# Autodesk Inventor assembly: Box Arm
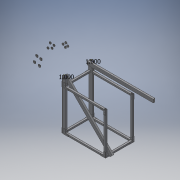
[picture p0: Inventor's stored thumbnail of the model, 180x180]
Saved by Autodesk Inventor 2018 (Build 220112000, 112)
## iProperties
Created: 2019-01-16
Part Number: Box Arm
Document SubType Name: Assembly
Designer: Gabriel
Author: Gabriel
## Documents named in this file (9)
- C:\Users\Gabriel\Documents\Drivebase Box Arm\Box Arm.iam
- C:\Users\Gabriel\Documents\Drivebase Box Arm\30in 1x1 Beam.ipt
- C:\Users\Gabriel\Documents\Drivebase Box Arm\25in 1x1 Beam.ipt
- C:\Users\Gabriel\Documents\Drivebase Box Arm\17in 1x1 Beam.ipt
- C:\Users\Gabriel\Documents\Drivebase Box Arm\23in 1x1 Beam.ipt
- C:\Users\Gabriel\Documents\Drivebase Box Arm\L gusset.ipt
- C:\Users\Gabriel\Documents\Drivebase Box Arm\34.48in Arm Bea.ipt
- C:\Users\Gabriel\Downloads\0_500_ID_x_1_125_OD_x_0_313_WD_Flanged_Bearing_217-2731.ipt
- C:\Users\Gabriel\Downloads\12t_Aluminum_Hub_Sprocket_35_Chain_1_2_Hex_Bore_217-2662.ipt
## Components (39 placed, 9 different names)
1. 30in 1x1 Beam:1 — Mate:13, Mate:14, Mate:37, Mate:38, Mate:74, Mate:75, Mate:81
2. 30in 1x1 Beam:2 — Mate:11, Mate:12, Mate:39, Mate:40, Mate:73, Mate:76, Mate:82
3. 25in 1x1 Beam:1 — Mate:57, Mate:58, Mate:59, Mate:60, Mate:65, Mate:66
4. 25in 1x1 Beam:2 — Mate:61, Mate:62, Mate:63, Mate:64, Mate:67, Mate:68
5. 25in 1x1 Beam:3 — Mate:29, Mate:30, Mate:53, Mate:54
6. 25in 1x1 Beam:4 — Mate:31, Mate:32, Mate:55, Mate:56
7. 17in 1x1 Beam:1 — Mate:69, Mate:70, Mate:71, Mate:72
8. 17in 1x1 Beam:2 — Mate:21, Mate:22, Mate:23, Mate:24
9. 23in 1x1 Beam:1 — Mate:43, Mate:44, Mate:49, Mate:50
10. 23in 1x1 Beam:2 — Mate:47, Mate:48, Mate:51, Mate:52
11. L gusset:1 — Mate:53, Mate:54, Mate:63, Mate:64
12. L gusset:4 — Mate:49, Mate:50, Mate:61, Mate:62
13. L gusset:5 — Mate:51, Mate:52, Mate:57, Mate:58
14. L gusset:7 — Mate:11, Mate:12, Mate:23, Mate:24
15. L gusset:9 — Mate:13, Mate:14, Mate:21, Mate:22
16. L gusset:11 — Mate:31, Mate:32, Mate:74, Mate:75
17. L gusset:12 — Mate:29, Mate:30, Mate:73, Mate:76
18. L gusset:13 — Mate:43, Mate:44
19. L gusset:14 — Mate:47, Mate:48
20. L gusset:15 — Mate:39, Mate:40, Mate:77, Mate:80
21. L gusset:16 — Mate:37, Mate:38, Mate:78, Mate:79
22. L gusset:17 — Mate:55, Mate:56, Mate:59, Mate:60
23. L gusset:18 — Mate:67, Mate:68, Mate:69, Mate:70
24. L gusset:19 — Mate:65, Mate:66, Mate:71, Mate:72
25. 34.48in Arm Beam:1 — Mate:82
26. 17in 1x1 Beam:3 — Mate:77, Mate:78, Mate:79, Mate:80
27. 34.48in Arm Bea:2 — Mate:81
28. 0_500_ID_x_1_125_OD_x_0_313_WD_Flanged_Bearing_217-2731:1
29. 0_500_ID_x_1_125_OD_x_0_313_WD_Flanged_Bearing_217-2731:2
30. 0_500_ID_x_1_125_OD_x_0_313_WD_Flanged_Bearing_217-2731:3
31. 0_500_ID_x_1_125_OD_x_0_313_WD_Flanged_Bearing_217-2731:4
32. 0_500_ID_x_1_125_OD_x_0_313_WD_Flanged_Bearing_217-2731:5
33. 0_500_ID_x_1_125_OD_x_0_313_WD_Flanged_Bearing_217-2731:6
34. 0_500_ID_x_1_125_OD_x_0_313_WD_Flanged_Bearing_217-2731:7
35. 0_500_ID_x_1_125_OD_x_0_313_WD_Flanged_Bearing_217-2731:8
36. 12t_Aluminum_Hub_Sprocket_35_Chain_1_2_Hex_Bore_217-2662:1
37. 12t_Aluminum_Hub_Sprocket_35_Chain_1_2_Hex_Bore_217-2662:2
38. 12t_Aluminum_Hub_Sprocket_35_Chain_1_2_Hex_Bore_217-2662:3
39. 12t_Aluminum_Hub_Sprocket_35_Chain_1_2_Hex_Bore_217-2662:4
## Relationships (54: Mate 54)
- Mate:11: 30in 1x1 Beam:2 ↔ L gusset:7
- Mate:12: 30in 1x1 Beam:2 ↔ L gusset:7
- Mate:13: 30in 1x1 Beam:1 ↔ L gusset:9
- Mate:14: 30in 1x1 Beam:1 ↔ L gusset:9
- Mate:21: 17in 1x1 Beam:2 ↔ L gusset:9
- Mate:22: 17in 1x1 Beam:2 ↔ L gusset:9
- Mate:23: 17in 1x1 Beam:2 ↔ L gusset:7
- Mate:24: 17in 1x1 Beam:2 ↔ L gusset:7
- Mate:29: 25in 1x1 Beam:3 ↔ L gusset:12
- Mate:30: 25in 1x1 Beam:3 ↔ L gusset:12
- Mate:31: 25in 1x1 Beam:4 ↔ L gusset:11
- Mate:32: 25in 1x1 Beam:4 ↔ L gusset:11
- Mate:37: 30in 1x1 Beam:1 ↔ L gusset:16
- Mate:38: 30in 1x1 Beam:1 ↔ L gusset:16
- Mate:39: 30in 1x1 Beam:2 ↔ L gusset:15
- Mate:40: 30in 1x1 Beam:2 ↔ L gusset:15
- Mate:43: 23in 1x1 Beam:1 ↔ L gusset:13
- Mate:44: 23in 1x1 Beam:1 ↔ L gusset:13
- Mate:47: 23in 1x1 Beam:2 ↔ L gusset:14
- Mate:48: 23in 1x1 Beam:2 ↔ L gusset:14
- Mate:49: 23in 1x1 Beam:1 ↔ L gusset:4
- Mate:50: 23in 1x1 Beam:1 ↔ L gusset:4
- Mate:51: 23in 1x1 Beam:2 ↔ L gusset:5
- Mate:52: 23in 1x1 Beam:2 ↔ L gusset:5
- Mate:53: 25in 1x1 Beam:3 ↔ L gusset:1
- Mate:54: 25in 1x1 Beam:3 ↔ L gusset:1
- Mate:55: 25in 1x1 Beam:4 ↔ L gusset:17
- Mate:56: 25in 1x1 Beam:4 ↔ L gusset:17
- Mate:57: 25in 1x1 Beam:1 ↔ L gusset:5
- Mate:58: 25in 1x1 Beam:1 ↔ L gusset:5
- Mate:59: 25in 1x1 Beam:1 ↔ L gusset:17
- Mate:60: 25in 1x1 Beam:1 ↔ L gusset:17
- Mate:61: 25in 1x1 Beam:2 ↔ L gusset:4
- Mate:62: 25in 1x1 Beam:2 ↔ L gusset:4
- Mate:63: 25in 1x1 Beam:2 ↔ L gusset:1
- Mate:64: 25in 1x1 Beam:2 ↔ L gusset:1
- Mate:65: 25in 1x1 Beam:1 ↔ L gusset:19
- Mate:66: 25in 1x1 Beam:1 ↔ L gusset:19
- Mate:67: 25in 1x1 Beam:2 ↔ L gusset:18
- Mate:68: 25in 1x1 Beam:2 ↔ L gusset:18
- Mate:69: 17in 1x1 Beam:1 ↔ L gusset:18
- Mate:70: 17in 1x1 Beam:1 ↔ L gusset:18
- Mate:71: 17in 1x1 Beam:1 ↔ L gusset:19
- Mate:72: 17in 1x1 Beam:1 ↔ L gusset:19
- Mate:73: 30in 1x1 Beam:2 ↔ L gusset:12
- Mate:74: 30in 1x1 Beam:1 ↔ L gusset:11
- Mate:75: 30in 1x1 Beam:1 ↔ L gusset:11
- Mate:76: 30in 1x1 Beam:2 ↔ L gusset:12
- Mate:77: L gusset:15 ↔ 17in 1x1 Beam:3
- Mate:78: L gusset:16 ↔ 17in 1x1 Beam:3
- Mate:79: L gusset:16 ↔ 17in 1x1 Beam:3
- Mate:80: L gusset:15 ↔ 17in 1x1 Beam:3
- Mate:81: 30in 1x1 Beam:1 ↔ 34.48in Arm Bea:2
- Mate:82: 30in 1x1 Beam:2 ↔ 34.48in Arm Beam:1
